# Autodesk Inventor assembly: 0_Entire_Assembly
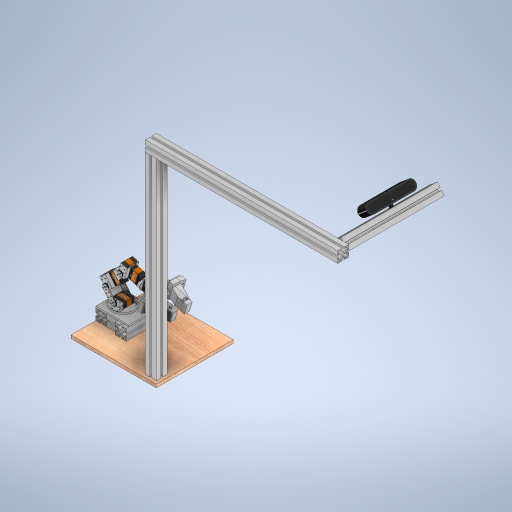
[picture p0: Inventor's stored thumbnail of the model, 512x512]
Saved by Autodesk Inventor 2024 (Build 280153000, 153)
## iProperties
Created: 2023-08-24
Part Number: 0_Entire_Assembly
Document SubType Name: Assembly
Designer: chanh
Author: chanh
## Documents named in this file (8)
- C:\Users\박동준\OneDrive - 연세대학교 (Yonsei University)\바탕 화면\박동준\대학생할\로봇\Humanoid\6축 매니퓰레이터\하드웨어\rh_plus_7_axis_robot_arm_hardware\Assembly\0_Entire_Assembly.iam
- C:\Users\박동준\OneDrive - 연세대학교 (Yonsei University)\바탕 화면\박동준\대학생할\로봇\Humanoid\6축 매니퓰레이터\하드웨어\rh_plus_7_axis_robot_arm_hardware\Assembly\2_Arm.iam
- C:\Users\박동준\OneDrive - 연세대학교 (Yonsei University)\바탕 화면\박동준\대학생할\로봇\Humanoid\6축 매니퓰레이터\하드웨어\rh_plus_7_axis_robot_arm_hardware\Assembly\3_Gripper.iam
- C:\Users\박동준\OneDrive - 연세대학교 (Yonsei University)\바탕 화면\박동준\대학생할\로봇\Humanoid\6축 매니퓰레이터\하드웨어\rh_plus_7_axis_robot_arm_hardware\Part\Other Parts\base_plate.ipt
- C:\Users\박동준\OneDrive - 연세대학교 (Yonsei University)\바탕 화면\박동준\대학생할\로봇\Humanoid\6축 매니퓰레이터\하드웨어\rh_plus_7_axis_robot_arm_hardware\Part\Other Parts\Aluminum_Profile_4040_test.ipt
- C:\Users\박동준\OneDrive - 연세대학교 (Yonsei University)\바탕 화면\박동준\대학생할\로봇\Humanoid\6축 매니퓰레이터\하드웨어\rh_plus_7_axis_robot_arm_hardware\Part\Other Parts\Aluminum_Profile_4040_test1.ipt
- C:\Users\박동준\OneDrive - 연세대학교 (Yonsei University)\바탕 화면\박동준\대학생할\로봇\Humanoid\6축 매니퓰레이터\하드웨어\rh_plus_7_axis_robot_arm_hardware\Part\Other Parts\Aluminum_Profile_4040_test2.ipt
- C:\Users\박동준\OneDrive - 연세대학교 (Yonsei University)\바탕 화면\박동준\대학생할\로봇\Humanoid\6축 매니퓰레이터\하드웨어\rh_plus_7_axis_robot_arm_hardware\Part\Other Parts\Astra_depth_camera.ipt
## Components (7 placed, 7 different names)
1. 2_Arm:1 [sub-assembly] — Flush:1, Flush:2, Flush:3, Rigid:1, Flush:4, Mate:1, Mate:2
2. 3_Gripper:1 [sub-assembly] — Rigid:1
3. base_plate:1 — Flush:4, Mate:1, Mate:2, Mate:3, Mate:4, Angle:3, Mate:8, Mate:9
4. Aluminum_Profile_4040_test:1 — Mate:6, Angle:4, Mate:7, Mate:8, Mate:9, Mate:10, Mate:11, Angle:5, Mate:12
5. Aluminum_Profile_4040_test1:1 — Flush:5, Flush:6, Mate:5, Mate:6, Angle:4, Mate:7
6. Aluminum_Profile_4040_test2:1 — Mate:3, Mate:4, Flush:5, Flush:6, Mate:5, Angle:3
7. Astra_depth_camera:1 — Mate:10, Mate:11, Angle:5, Mate:12
## Relationships (22: Mate 12, Flush 6, Angle 3, WeldJoint 1)
- Flush:1: 2_Arm:1
- Flush:2: 2_Arm:1
- Flush:3: 2_Arm:1
- Rigid:1 [WeldJoint]: 2_Arm:1 ↔ 3_Gripper:1
- Flush:4: 2_Arm:1 ↔ base_plate:1
- Mate:1: 2_Arm:1 ↔ base_plate:1
- Mate:2: 2_Arm:1 ↔ base_plate:1
- Mate:3: base_plate:1 ↔ Aluminum_Profile_4040_test2:1
- Mate:4: base_plate:1 ↔ Aluminum_Profile_4040_test2:1
- Flush:5: Aluminum_Profile_4040_test1:1 ↔ Aluminum_Profile_4040_test2:1
- Flush:6: Aluminum_Profile_4040_test1:1 ↔ Aluminum_Profile_4040_test2:1
- Mate:5: Aluminum_Profile_4040_test1:1 ↔ Aluminum_Profile_4040_test2:1
- Angle:3 (0 deg): base_plate:1 ↔ Aluminum_Profile_4040_test2:1
- Mate:6: Aluminum_Profile_4040_test:1 ↔ Aluminum_Profile_4040_test1:1
- Angle:4 (140 deg): Aluminum_Profile_4040_test:1 ↔ Aluminum_Profile_4040_test1:1
- Mate:7: Aluminum_Profile_4040_test:1 ↔ Aluminum_Profile_4040_test1:1
- Mate:8 (720 mm): base_plate:1 ↔ Aluminum_Profile_4040_test:1
- Mate:9 (620 mm): base_plate:1 ↔ Aluminum_Profile_4040_test:1
- Mate:10: Aluminum_Profile_4040_test:1 ↔ Astra_depth_camera:1
- Mate:11 (4.5 mm): Aluminum_Profile_4040_test:1 ↔ Astra_depth_camera:1
- Angle:5 (0 deg): Aluminum_Profile_4040_test:1 ↔ Astra_depth_camera:1
- Mate:12 (-150 mm): Aluminum_Profile_4040_test:1 ↔ Astra_depth_camera:1
